# Autodesk Inventor assembly: Fixture Assembly
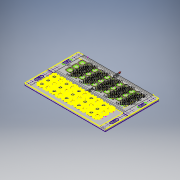
[picture p0: Inventor's stored thumbnail of the model, 180x180]
Saved by Autodesk Inventor 2016 (Build 200138000, 138)
## iProperties
Created: 2016-04-08
Part Number: Fixture Assembly
Document SubType Name: Assembly
Designer: Sam Clay
Author: Sam Clay
## Documents named in this file (7)
- Z:\enclosure\inventor\Fixture Assembly.iam
- Z:\enclosure\inventor\Fixture Base.ipt
- Z:\enclosure\inventor\Case Top.ipt
- Z:\enclosure\inventor\Case Bottom.ipt
- Z:\enclosure\inventor\Case Top Fixture.ipt
- Z:\enclosure\inventor\Case Bottom Fixture.ipt
- Z:\enclosure\inventor\Clamps\Desatco Clamp 205-S.iam
## Components (63 placed, 6 different names)
1. Fixture Base:1 — Planar:6, Mate:4, Mate:5, Bottom contour planar, Angle:1, Planar:12, Planar:13
2. Desatco Clamp 205-S:1 [sub-assembly] — Planar:12
3. Desatco Clamp 205-S:2 [sub-assembly] — Planar:13
4. Case Bottom:1 — Planar:6, Mate top pocket shell, Mate side pocket shell
5. Case Bottom:2
6. Case Bottom:3
7. Case Bottom:4
8. Case Bottom:5
9. Case Bottom:6
10. Case Bottom:7
11. Case Bottom:8
12. Case Bottom:9
13. Case Bottom:10
14. Case Bottom:11
15. Case Bottom:12
16. Case Bottom:13
17. Case Bottom:14
18. Case Bottom:15
19. Case Top:2 — Mate:4, Mate:5, Mate side pocket shell, Mate top pocket shell
20. Case Top:3
21. Case Top:4
22. Case Top:5
23. Case Top:6
24. Case Top:7
25. Case Top:8
26. Case Top:9
27. Case Top:10
28. Case Top:11
29. Case Top:12
30. Case Top:13
31. Case Top:14
32. Case Top:15
33. Case Top:16
34. Case Top Fixture:1 — Mate:8, Mate:9
35. Case Top Fixture:2
36. Case Top Fixture:3
37. Case Top Fixture:4
38. Case Top Fixture:5
39. Case Top Fixture:6
40. Case Top Fixture:7
41. Case Top Fixture:8
42. Case Top Fixture:9
43. Case Top Fixture:10
44. Case Top Fixture:11
45. Case Top Fixture:12
46. Case Top Fixture:13
47. Case Top Fixture:14
48. Case Top Fixture:15
49. Case Bottom Fixture:1 — Bottom contour planar, Angle:1, Mate:8, Mate:9
50. Case Bottom Fixture:2
51. Case Bottom Fixture:3
52. Case Bottom Fixture:4
53. Case Bottom Fixture:5
54. Case Bottom Fixture:6
55. Case Bottom Fixture:7
56. Case Bottom Fixture:8
57. Case Bottom Fixture:9
58. Case Bottom Fixture:10
59. Case Bottom Fixture:11
60. Case Bottom Fixture:12
61. Case Bottom Fixture:13
62. Case Bottom Fixture:14
63. Case Bottom Fixture:15
## Component patterns: (15 elements, first: Case Bottom:1), (15 elements, first: Case Top:2), (15 elements, first: Case Top Fixture:1), (15 elements, first: Case Bottom Fixture:1)
## Relationships (11: Mate 6, PlanarJoint 4, Angle 1)
- Planar:6: Fixture Base:1 ↔ Case Bottom:1
- Mate:4 (2.54 mm): Fixture Base:1 ↔ Case Top:2
- Mate:5 (6.604 mm): Fixture Base:1 ↔ Case Top:2
- Mate top pocket shell: Case Bottom:1 ↔ Case Top:2
- Mate side pocket shell (6.604 mm): Case Bottom:1 ↔ Case Top:2
- Bottom contour planar [PlanarJoint] (16.51 mm): Fixture Base:1 ↔ Case Bottom Fixture:1
- Angle:1 (0 deg): Fixture Base:1 ↔ Case Bottom Fixture:1
- Mate:8 (6.604 mm): Case Top Fixture:1 ↔ Case Bottom Fixture:1
- Mate:9: Case Top Fixture:1 ↔ Case Bottom Fixture:1
- Planar:12: Fixture Base:1 ↔ Desatco Clamp 205-S:1
- Planar:13: Fixture Base:1 ↔ Desatco Clamp 205-S:2
